# Autodesk Inventor assembly: Slewing
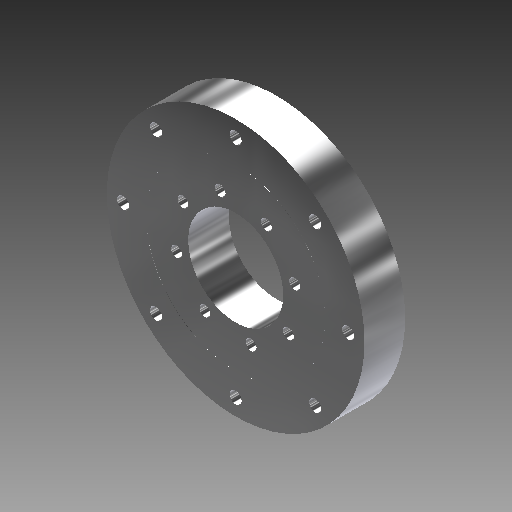
[picture p0: Inventor's stored thumbnail of the model, 512x512]
Saved by Autodesk Inventor 2017 (Build 210142000, 142)
## iProperties
Created: 2019-08-28
Part Number: Slewing
Document SubType Name: Assembly
Designer: Dell
Author: Dell
## Documents named in this file (3)
- C:\Users\Dell\Documents\GitHub\tr2\Actuator 1.5\Slewing.iam
- C:\Users\Dell\Documents\GitHub\tr2\Actuator 1.5\Slewing A.ipt
- C:\Users\Dell\Documents\GitHub\tr2\Actuator 1.5\Slewing B.ipt
## Components (2 placed, 2 different names)
1. Slewing A:1 — Mate:1, Flush:1
2. Slewing B:1 — Mate:1, Flush:1
## Relationships (2: Mate 1, Flush 1)
- Mate:1: Slewing A:1 ↔ Slewing B:1
- Flush:1: Slewing A:1 ↔ Slewing B:1
